# Autodesk Inventor assembly: Tape Measure Bracket Assembly V4
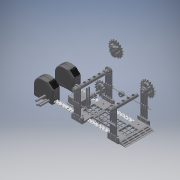
[picture p0: Inventor's stored thumbnail of the model, 180x180]
Saved by Autodesk Inventor 2019 (Build 230136000, 136)
## iProperties
Created: 2018-11-08
Part Number: Tape Measure Bracket Assembly V4
Document SubType Name: Assembly
Designer: Ashley
Author: Ashley
## Documents named in this file (16)
- C:\Users\Ashley\Desktop\repositories\design\inventor\2018-2019\Tape Measure Braket\Version Four\Tape Measure Bracket Assembly V4.iam
- C:\Users\Ashley\Desktop\repositories\design\inventor\2018-2019\Tape Measure Braket\Version Four\Bracket Bottom V4.ipt
- C:\Users\Ashley\Desktop\repositories\design\inventor\2018-2019\Tape Measure Braket\Tape Measure\Tape Measure Edited.iam
- C:\Users\Ashley\Desktop\repositories\design\inventor\2018-2019\Tape Measure Braket\Version Four\Side V4.ipt
- C:\Users\Ashley\Desktop\repositories\design\inventor\Imported Components\goBilda\Bearing6mmID.ipt
- C:\Users\Ashley\Desktop\repositories\design\inventor\2018-2019\Tape Measure Braket\Version Four\SpinnerV4.ipt
- C:\Users\Ashley\Desktop\repositories\design\inventor\Imported Components\goBilda\Collar6mm\SetScrewCollar6mmboreassembly.iam
- C:\Users\Ashley\Desktop\repositories\design\inventor\2018-2019\Tape Measure Braket\Finished Parts\2mmAxel.ipt
- C:\Users\Ashley\Desktop\repositories\design\inventor\Imported Components\goBilda\CampingHub\ClampingHub assembly.iam
- C:\Users\Ashley\Desktop\repositories\design\inventor\Imported Components\goBilda\8mmPlasticPitchSproket.ipt
- C:\Users\Ashley\Desktop\repositories\design\inventor\2018-2019\Tape Measure Braket\Version Two\Braket Top V2.ipt
- C:\Users\Ashley\Desktop\repositories\design\inventor\Imported Components\REV\Motors and Servos\Rev_Servo.iam
- C:\Users\Ashley\Desktop\repositories\design\inventor\2018-2019\Tape Measure Braket\Version Three\Servo Locks V3.ipt
- C:\Users\Ashley\Desktop\repositories\design\inventor\Imported Components\goBilda\Servo To Shaft\ServoToShaftCoupler.iam
- C:\Users\Ashley\Desktop\repositories\design\inventor\Imported Components\goBilda\DShaft40mm.ipt
- C:\Users\Ashley\Desktop\repositories\design\inventor\Imported Components\goBilda\DShaft30mm.ipt
## Components (41 placed, 32 different names)
1. Bracket Bottom — Mate:1, Mate:4, Mate:5, Mate:6, Mate:7, Mate:9, Mate:10
2. Tape Measure Right [sub-assembly]
3. Tape Measure Left [sub-assembly]
4. Back Right Side — Mate:9, Mate:11
5. Front Right Side — Mate:1, Insert:2, Insert:11
6. Front Left Side — Insert:3, Insert:10
7. Back Right Bearing — Mate:11, Mate:12
8. Front Right Bearing — Insert:2
9. Front Left Beaing — Insert:3
10. Front Left BEaring — Insert:23
11. Back Spinner
12. Front Spinner
13. Front Right Collar [sub-assembly]
14. Front Left Collar [sub-assembly]
15. Back Left Collar [sub-assembly]
16. Back Right Collar [sub-assembly]
17. Left axel — Insert:10
18. Right Axel — Insert:11
19. Front Sproket — Insert:12
20. Front Claming Hub [sub-assembly] — Insert:12
21. Back Sproket — Insert:37
22. Back Clamping Hub [sub-assembly] — Insert:37
23. Side V4:4 — Insert:23, Mate:10
24. Braket Top V2:1 — Mate:5
25. Braket Top V2:2 — Mate:4
26. Braket Top V2:3
27. Braket Top V2:4
28. Rev_Servo:1 [sub-assembly] — Mate:8, Insert:24
29. Servo Locks V3:1 — Mate:7, Mate:8
30. Servo Locks V3:2 — Mate:6
31. ServoToShaftCoupler:1 [sub-assembly] — Insert:24, Insert:25
32. DShaft40mm:1 — Insert:25, Insert:27
33. 8mmPlasticPitchSproket:3 — Insert:28
34. ClampingHub assembly:3 [sub-assembly] — Insert:27, Insert:28
35. DShaft30mm:2 — Mate:12
36. DShaft30mm:3
37. DShaft30mm:4
38. DShaft30mm:5
39. SetScrewCollar6mmboreassembly:8 [sub-assembly]
40. SetScrewCollar6mmboreassembly:9 [sub-assembly]
41. SetScrewCollar6mmboreassembly:10 [sub-assembly]
## Relationships (23: Insert 13, Mate 10)
- Mate:1: Bracket Bottom ↔ Front Right Side
- Insert:2: Front Right Side ↔ Front Right Bearing
- Insert:3: Front Left Side ↔ Front Left Beaing
- Insert:10 (-30 mm): Front Left Side ↔ Left axel
- Insert:11 (-30 mm): Front Right Side ↔ Right Axel
- Insert:12 (-1 mm): Front Sproket ↔ Front Claming Hub
- [Insert] (-1 mm): Back Sproket ↔ Back Clamping Hub
- Insert:23: Front Left BEaring ↔ Side V4:4
- Mate:4: Bracket Bottom ↔ Braket Top V2:2
- Mate:5: Bracket Bottom ↔ Braket Top V2:1
- Mate:6: Bracket Bottom ↔ Servo Locks V3:2
- Mate:7: Bracket Bottom ↔ Servo Locks V3:1
- Mate:8: Rev_Servo:1 ↔ Servo Locks V3:1
- Insert:24 (-3.5 mm): Rev_Servo:1 ↔ ServoToShaftCoupler:1
- Insert:25 (30 mm): ServoToShaftCoupler:1 ↔ DShaft40mm:1
- [Insert] (-1 mm): 8mmPlasticPitchSproket:3 ↔ ClampingHub assembly:3
- Insert:27 (3 mm): DShaft40mm:1 ↔ ClampingHub assembly:3
- Insert:28 (-1 mm): 8mmPlasticPitchSproket:3 ↔ ClampingHub assembly:3
- Mate:9: Bracket Bottom ↔ Back Right Side
- Mate:10: Bracket Bottom ↔ Side V4:4
- Mate:11: Back Right Side ↔ Back Right Bearing
- Insert:37 (-1 mm): Back Sproket ↔ Back Clamping Hub
- Mate:12: Back Right Bearing ↔ DShaft30mm:2
## Named parameters: d26_d25 = -1 mm, d46_d26_d25 = -1 mm
